# Autodesk Inventor assembly: Gamepad_Right
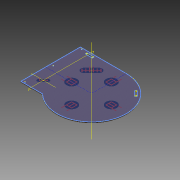
[picture p0: Inventor's stored thumbnail of the model, 180x180]
Saved by Autodesk Inventor 2014 SP1 (Build 180222100, 222)
## iProperties
Created: 2014-02-22
Part Number: Gamepad_Right
Document SubType Name: Assembly
Designer: tuleu
Author: tuleu
## Documents named in this file (6)
- C:\Users\tuleu\Documents\giant-snes-gamepad\cad\Gamepad_Right.iam
- C:\Users\tuleu\Documents\giant-snes-gamepad\cad\Trigger_Cell.iam
- C:\Users\tuleu\Documents\giant-snes-gamepad\cad\Start_Cell.iam
- C:\Users\tuleu\Documents\giant-snes-gamepad\cad\Circle_Cell.iam
- C:\Users\tuleu\Documents\giant-snes-gamepad\cad\Base_Right.ipt
- C:\Users\tuleu\Documents\giant-snes-gamepad\cad\Foam_Right.ipt
## Components (8 placed, 5 different names)
1. Trigger_Cell:1 [sub-assembly]
2. Start_Cell:1 [sub-assembly]
3. Circle_Cell:1 [sub-assembly]
4. Circle_Cell:2 [sub-assembly]
5. Circle_Cell:3 [sub-assembly]
6. Circle_Cell:4 [sub-assembly]
7. Base_Right:1 — Flush:1, Flush:2
8. Foam_Right:1 — Flush:1, Flush:2
## Relationships (19: Mate 17, Flush 2)
- [Mate]: Circle_Cell:1 ↔ Circle_Cell:3
- [Mate]: Circle_Cell:2 ↔ Circle_Cell:4
- [Mate]: Trigger_Cell:1 ↔ Base_Right:1
- [Mate]: Trigger_Cell:1 ↔ Base_Right:1
- [Mate] (-400 mm): Trigger_Cell:1 ↔ Base_Right:1
- [Mate]: Start_Cell:1 ↔ Base_Right:1
- [Mate]: Start_Cell:1 ↔ Base_Right:1
- [Mate]: Circle_Cell:1 ↔ Base_Right:1
- [Mate]: Circle_Cell:2 ↔ Base_Right:1
- [Mate]: Circle_Cell:3 ↔ Base_Right:1
- [Mate]: Circle_Cell:4 ↔ Base_Right:1
- [Mate]: Circle_Cell:1 ↔ Base_Right:1
- [Mate]: Circle_Cell:2 ↔ Base_Right:1
- [Mate] (-280 mm): Circle_Cell:1 ↔ Base_Right:1
- [Mate] (-280 mm): Circle_Cell:3 ↔ Base_Right:1
- [Mate] (-280 mm): Circle_Cell:2 ↔ Base_Right:1
- [Mate] (-280 mm): Circle_Cell:4 ↔ Base_Right:1
- Flush:1: Base_Right:1 ↔ Foam_Right:1
- Flush:2: Base_Right:1 ↔ Foam_Right:1
